# Autodesk Inventor assembly: output
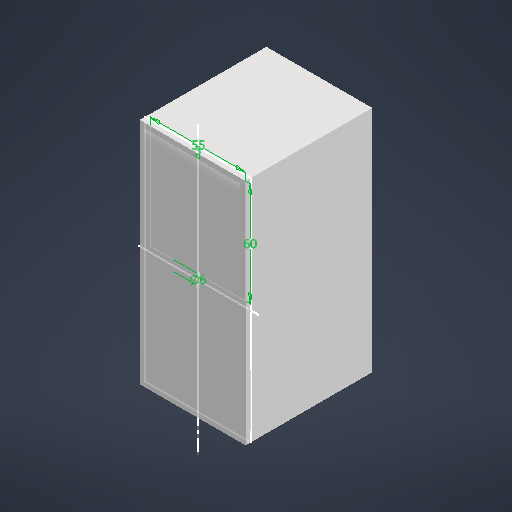
[picture p0: Inventor's stored thumbnail of the model, 512x512]
Saved by Autodesk Inventor 2025.3 (Build 293356030, 356C)
## iProperties
Created: 2025-12-14
Part Number: output
Document SubType Name: Assembly
Designer: 陳泓任
Author: 陳泓任
## Documents named in this file (3)
- D:\3D-model-temp\self-learning\output.iam
- D:\3D-model-temp\self-learning\frame.ipt
- D:\3D-model-temp\self-learning\door.ipt
## Components (2 placed, 2 different names)
1. frame:1 — 貼合:1, 貼合:2
2. door:1 — 貼合:1, 貼合:2
## Relationships (2: Mate 2)
- 貼合:1 [Mate]: frame:1 ↔ door:1
- 貼合:2 [Mate]: frame:1 ↔ door:1
